# Autodesk Inventor assembly: OREJA_DE_IZAJE
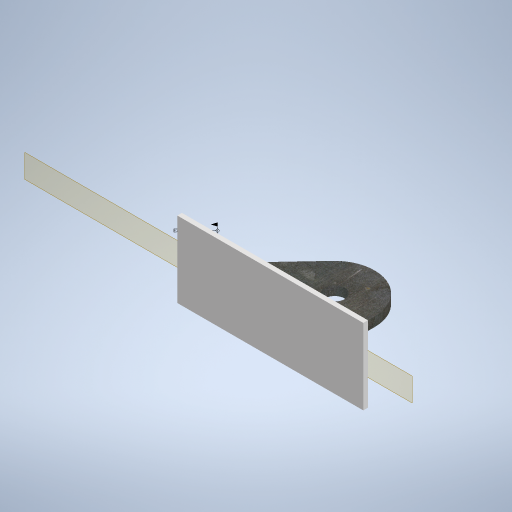
[picture p0: Inventor's stored thumbnail of the model, 512x512]
Saved by Autodesk Inventor 2023 (Build 270158000, 158)
## iProperties
RuleStatus: InUse
AfterDocOpen0: CLICK_DERECHO_EJECUTAR_REGLA
Created: 2023-06-02
Part Number: OREJA_DE_IZAJE
Document SubType Name: Conjunto soldado
Designer: NELSON ORTIZ
Weld Material: Acero ASTM A500 Gr. C.
Mass: 32741.8 g
Surface Area: 11080.7 cm^2
Volume: 10481.4 cm^3
Density: 3.12381 g/cm^3
Author: NELSON ORTIZ
## Documents named in this file (3)
- C:\Users\norti\OneDrive\PLANOS\OREJA DE IZAJE\OREJA_DE_IZAJE.iam
- C:\Users\norti\OneDrive\PLANOS\OREJA DE IZAJE\OREJA_DE_IZAJE.ipt
- C:\Users\norti\OneDrive\PLANOS\OREJA DE IZAJE\LAMINA_PARA_OREJA_DE_IZAJE.ipt
## Components (2 placed, 2 different names)
1. OREJA_DE_IZAJE:1 — Nivelación:1, Nivelación:2, Nivelación:3, Coincidencia:1
2. LAMINA_PARA_OREJA_DE_IZAJE:1 — Nivelación:1, Nivelación:2, Nivelación:3, Coincidencia:1
## Relationships (4: Flush 3, Mate 1)
- Nivelación:1 [Flush]: OREJA_DE_IZAJE:1 ↔ LAMINA_PARA_OREJA_DE_IZAJE:1
- Nivelación:2 [Flush] (-50 mm): OREJA_DE_IZAJE:1 ↔ LAMINA_PARA_OREJA_DE_IZAJE:1
- Nivelación:3 [Flush] (-50 mm): OREJA_DE_IZAJE:1 ↔ LAMINA_PARA_OREJA_DE_IZAJE:1
- Coincidencia:1 [Mate]: OREJA_DE_IZAJE:1 ↔ LAMINA_PARA_OREJA_DE_IZAJE:1
## Named parameters: Grosor = 14 mm, areadesarrollo = 1537, anchodesarrollo = 290 mm, largodesarrollo = 530 mm, L = 180 mm, epl = 14 mm, h_ = 60 mm, r = 60 mm, hole = 30 mm, hole_gr = 25.4 mm, a = 7 mm, b = 20 mm, eb = 7 mm, ton = 6, peso = 1.6, grillete = 0.875 mm, iTrigger0 = 1
note: some values were not read from the file. Shown as the stored number, unit unknown: "areadesarrollo", "peso".
